# Autodesk Inventor assembly: UM gantry
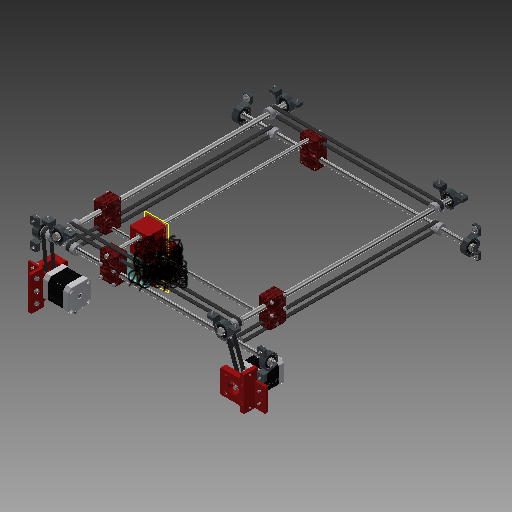
[picture p0: Inventor's stored thumbnail of the model, 512x512]
Saved by Autodesk Inventor 2018.1 (Build 221171000, 171)
## iProperties
Part Number: UM gantry
Material: Generisch
Document SubType Name: Assembly
Designer: Till
Author: Till
## Documents named in this file (18)
- C:\Users\tillm\Dropbox\DIY\CoreBot\UM gantry.iam
- C:\Users\tillm\Dropbox\DIY\CAD\KP08\KP08.iam
- C:\Users\tillm\Dropbox\DIY\CoreBot\CAD Parts\8mm hardened rod.ipt
- C:\Users\tillm\Dropbox\DIY\CoreBot\sliding block.iam
- C:\Users\tillm\Dropbox\DIY\CoreBot\CAD Parts\DriveLine 8x400mm.ipt
- C:\Users\tillm\Dropbox\DIY\CoreBot\CAD Parts\DriveLine 8x350mm.ipt
- C:\Users\tillm\Dropbox\DIY\CoreBot\CAD Parts\1166-B2P-A.ipt
- C:\Users\tillm\Dropbox\DIY\CoreBot\Y belt.ipt
- C:\Users\tillm\Dropbox\DIY\CoreBot\X belt.ipt
- C:\Users\tillm\Dropbox\DIY\CoreBot\CAD Parts\NEMA 17.ipt
- C:\Users\tillm\Dropbox\DIY\CoreBot\CAD Parts\GT2_20teeth_pulley.ipt
- C:\Users\tillm\Dropbox\DIY\CoreBot\CAD Parts\1167-B2P-A (2).ipt
- C:\Users\tillm\Dropbox\DIY\CoreBot\motor belt.ipt
- C:\Users\tillm\Dropbox\DIY\CoreBot\Y motor mount.ipt
- C:\Users\tillm\Dropbox\DIY\CoreBot\X motor mount.ipt
- C:\Users\tillm\Dropbox\DIY\CoreBot\M3 x 10.ipt
- C:\Users\tillm\Dropbox\DIY\CoreBot\CAD Parts\item_0_0_616_29_6rrjpzm9kai2q6ysfss7799ws.ipt
- C:\Users\tillm\Dropbox\DIY\CoreBot\Hotend 2.2.iam
## Components (56 placed, 27 different names)
1. DriveLine 8x400mm:1 — Passend:20, Fluchtend:23, Passend:104
2. DriveLine 8x350mm:1 — Passend:21, Fluchtend:24
3. Hotend 2.2:3 [sub-assembly] — Passend:104, Winkel:12, Fluchtend:106
4. X front right [sub-assembly] — Fluchtend:7, Passend:4, Passend:5, Fluchtend:8, Fluchtend:9, Passend:6, Passend:7, Fluchtend:10, Fluchtend:11, Fluchtend:14, Passend:9, Fluchtend:16, Winkel:3
5. X front left [sub-assembly] — Passend:7, Fluchtend:10, Fluchtend:11, Fluchtend:12, Fluchtend:13, Passend:8, Fluchtend:15, Passend:10, Winkel:4
6. X back right [sub-assembly] — Fluchtend:8, Fluchtend:9, Passend:6, Passend:11, Fluchtend:17, Winkel:7, Fluchtend:43
7. X back left [sub-assembly] — Fluchtend:12, Fluchtend:13, Passend:8
8. Y front right [sub-assembly] — Fluchtend:1, Passend:1, Fluchtend:2, Passend:2, Fluchtend:3, Fluchtend:6, Fluchtend:7, Passend:4, Passend:5, Passend:12, Fluchtend:18, Winkel:1, Passend:71, Fluchtend:42
9. Y front left [sub-assembly] — Passend:2, Fluchtend:3, Fluchtend:4, Passend:3, Fluchtend:5, Fluchtend:6, Passend:13, Fluchtend:19
10. Y back right [sub-assembly] — Fluchtend:1, Passend:1, Fluchtend:2, Fluchtend:44
11. Y back left [sub-assembly] — Fluchtend:4, Passend:3, Fluchtend:5
12. X front — Passend:10, Fluchtend:16, Passend:17, Passend:28, Passend:29, Passend:79
13. X back — Passend:11, Fluchtend:17, Passend:16, Passend:27, Passend:48
14. Y right — Passend:12, Fluchtend:18, Passend:14, Passend:24, Passend:31, Passend:57
15. Y left — Passend:13, Fluchtend:19, Passend:15, Passend:23, Passend:26
16. sliding block:1 [sub-assembly] — Passend:17, Winkel:1, Winkel:2, Passend:21, Fluchtend:24, Winkel:8, Winkel:9, Fluchtend:45, Winkel:11, Passend:78
17. sliding block:2 [sub-assembly] — Passend:16, Winkel:2, Fluchtend:30, Winkel:9, Fluchtend:45, Winkel:10, Winkel:12, Fluchtend:106
18. sliding block:3 [sub-assembly] — Passend:15, Winkel:4, Fluchtend:47, Passend:80
19. sliding block:4 [sub-assembly] — Passend:14, Winkel:3, Passend:20, Fluchtend:23, Fluchtend:28, Fluchtend:47
20. Y belt:1 — Fluchtend:35, Winkel:6, Passend:79, Passend:80
21. Y belt:2 — Passend:35, Winkel:7, Passend:36, Passend:49
22. X belt:1 — Passend:37, Passend:40, Winkel:11, Passend:78
23. X belt:2 — Passend:38, Passend:41, Winkel:10
24. 1167-B2P-A (2):1 — Passend:48, Passend:49, Passend:51, Passend:54
25. 1166-B2P-A:1 — Passend:26, Fluchtend:30, Passend:41, Fluchtend:36
26. 1166-B2P-A:3 — Passend:27, Fluchtend:27, Fluchtend:35
27. 1166-B2P-A:4 — Passend:24, Fluchtend:34, Passend:37, Passend:40
28. 1166-B2P-A:5 — Passend:57, Passend:59, Passend:58
29. 1166-B2P-A:6 — Passend:23, Fluchtend:34
30. 1166-B2P-A:7 — Passend:28, Fluchtend:27
31. 1166-B2P-A:8 — Passend:29, Fluchtend:28, Passend:35, Passend:36
32. 1166-B2P-A:9 — Passend:31, Passend:38, Fluchtend:36
33. item_0_0_616_29_6rrjpzm9kai2q6ysfss7799ws:5 — Fluchtend:56, Passend:103
34. item_0_0_616_29_6rrjpzm9kai2q6ysfss7799ws:6 — Fluchtend:56, Passend:99, Passend:100
35. item_0_0_616_29_6rrjpzm9kai2q6ysfss7799ws:8 — Passend:101
36. M3 x 10:1 — Fluchtend:48, Passend:84, Passend:85
37. M3 x 10:2 — Fluchtend:48, Passend:86
38. M3 x 10:3 — Fluchtend:49, Passend:83
39. M3 x 10:4 — Fluchtend:49, Passend:81, Passend:82
40. GT2_20teeth_pulley:2 — Passend:42, Passend:55, Passend:65
41. NEMA 17:2 — Passend:42, Passend:75, Passend:76, Passend:77
42. motor belt:1 — Passend:51, Passend:54, Passend:55, Passend:65
43. X motor mount:1 — Passend:75, Fluchtend:43, Fluchtend:44, Passend:76, Passend:77, Passend:81, Passend:82, Passend:83, Passend:84, Passend:85, Passend:86, Passend:99, Passend:100, Passend:101, Passend:103
44. item_0_0_616_29_6rrjpzm9kai2q6ysfss7799ws:1 — Fluchtend:55, Passend:94, Passend:95
45. item_0_0_616_29_6rrjpzm9kai2q6ysfss7799ws:2 — Fluchtend:54, Fluchtend:55, Passend:96
46. item_0_0_616_29_6rrjpzm9kai2q6ysfss7799ws:3 — Fluchtend:53, Fluchtend:54, Passend:97
47. item_0_0_616_29_6rrjpzm9kai2q6ysfss7799ws:4 — Fluchtend:53, Passend:98
48. M3 x 10:5 — Fluchtend:50, Passend:93
49. M3 x 10:6 — Fluchtend:50, Passend:91, Passend:92
50. M3 x 10:7 — Fluchtend:51, Passend:89
51. M3 x 10:8 — Fluchtend:51, Fluchtend:52, Passend:90
52. M3 x 10:9 — Fluchtend:52, Passend:87, Passend:88
53. Y motor mount:1 — Passend:71, Fluchtend:42, Passend:72, Passend:73, Passend:74, Winkel:8, Passend:87, Passend:88, Passend:89, Passend:90, Passend:91, Passend:92, Passend:93, Passend:94, Passend:95, Passend:96, Passend:97, Passend:98
54. motor belt:2 — Passend:56, Passend:59, Passend:58, Passend:69
55. GT2_20teeth_pulley:1 — Passend:43, Passend:56, Passend:69
56. NEMA 17:1 — Passend:43, Passend:72, Passend:73, Passend:74
## Relationships (131: Mate 78, Flush 42, Angle 11)
- Fluchtend:1 [Flush]: Y front right ↔ Y back right
- Passend:1 [Mate] (407 mm): Y front right ↔ Y back right
- Fluchtend:2 [Flush]: Y front right ↔ Y back right
- Passend:2 [Mate] (-400 mm): Y front right ↔ Y front left
- Fluchtend:3 [Flush]: Y front right ↔ Y front left
- Fluchtend:4 [Flush]: Y front left ↔ Y back left
- Passend:3 [Mate] (410 mm): Y front left ↔ Y back left
- Fluchtend:5 [Flush]: Y front left ↔ Y back left
- Fluchtend:6 [Flush]: Y front right ↔ Y front left
- Fluchtend:7 [Flush] (-20.1 mm): X front right ↔ Y front right
- Passend:4 [Mate] (23.6 mm): X front right ↔ Y front right
- Passend:5 [Mate] (3.5 mm): X front right ↔ Y front right
- Fluchtend:8 [Flush]: X front right ↔ X back right
- Fluchtend:9 [Flush]: X front right ↔ X back right
- Passend:6 [Mate] (-359.8 mm): X front right ↔ X back right
- Passend:7 [Mate] (407 mm): X front right ↔ X front left
- Fluchtend:10 [Flush]: X front right ↔ X front left
- Fluchtend:11 [Flush]: X front right ↔ X front left
- Fluchtend:12 [Flush]: X front left ↔ X back left
- Fluchtend:13 [Flush]: X front left ↔ X back left
- Passend:8 [Mate] (-359.8 mm): X front left ↔ X back left
- Fluchtend:14 [Flush]: X front right
- Passend:9 [Mate]: X front right
- Fluchtend:15 [Flush]: X front left
- Passend:10 [Mate]: X front left ↔ X front
- Fluchtend:16 [Flush]: X front right ↔ X front
- Passend:11 [Mate]: X back right ↔ X back
- Fluchtend:17 [Flush]: X back right ↔ X back
- Passend:12 [Mate]: Y front right ↔ Y right
- Fluchtend:18 [Flush]: Y front right ↔ Y right
- Passend:13 [Mate]: Y front left ↔ Y left
- Fluchtend:19 [Flush]: Y front left ↔ Y left
- Passend:14 [Mate]: Y right ↔ sliding block:4
- Passend:15 [Mate]: Y left ↔ sliding block:3
- Passend:16 [Mate]: X back ↔ sliding block:2
- Passend:17 [Mate]: X front ↔ sliding block:1
- Winkel:1 [Angle] (0 deg): Y front right ↔ sliding block:1
- Winkel:2 [Angle] (0 deg): sliding block:1 ↔ sliding block:2
- Winkel:3 [Angle] (0 deg): X front right ↔ sliding block:4
- Winkel:4 [Angle] (0 deg): X front left ↔ sliding block:3
- Passend:20 [Mate]: DriveLine 8x400mm:1 ↔ sliding block:4
- Fluchtend:23 [Flush] (-5 mm): DriveLine 8x400mm:1 ↔ sliding block:4
- Passend:21 [Mate]: DriveLine 8x350mm:1 ↔ sliding block:1
- Fluchtend:24 [Flush] (-5 mm): DriveLine 8x350mm:1 ↔ sliding block:1
- Passend:23 [Mate]: Y left ↔ 1166-B2P-A:6
- Passend:24 [Mate]: Y right ↔ 1166-B2P-A:4
- Passend:26 [Mate]: Y left ↔ 1166-B2P-A:1
- Passend:27 [Mate]: X back ↔ 1166-B2P-A:3
- Passend:28 [Mate]: X front ↔ 1166-B2P-A:7
- Passend:29 [Mate]: X front ↔ 1166-B2P-A:8
- Passend:31 [Mate]: Y right ↔ 1166-B2P-A:9
- Fluchtend:34 [Flush]: 1166-B2P-A:4 ↔ 1166-B2P-A:6
- Fluchtend:27 [Flush]: 1166-B2P-A:3 ↔ 1166-B2P-A:7
- Fluchtend:28 [Flush]: sliding block:4 ↔ 1166-B2P-A:8
- Fluchtend:30 [Flush]: sliding block:2 ↔ 1166-B2P-A:1
- Fluchtend:35 [Flush]: Y belt:1 ↔ 1166-B2P-A:3
- Winkel:6 [Angle] (0 deg): Y belt:1
- Passend:35 [Mate]: Y belt:2 ↔ 1166-B2P-A:8
- Winkel:7 [Angle] (0 deg): X back right ↔ Y belt:2
- Passend:36 [Mate]: Y belt:2 ↔ 1166-B2P-A:8
- Passend:37 [Mate]: X belt:1 ↔ 1166-B2P-A:4
- Passend:38 [Mate]: X belt:2 ↔ 1166-B2P-A:9
- Passend:41 [Mate]: X belt:2 ↔ 1166-B2P-A:1
- Passend:40 [Mate]: X belt:1 ↔ 1166-B2P-A:4
- Fluchtend:36 [Flush]: 1166-B2P-A:1 ↔ 1166-B2P-A:9
- Passend:42 [Mate]: GT2_20teeth_pulley:2 ↔ NEMA 17:2
- Passend:43 [Mate]: GT2_20teeth_pulley:1 ↔ NEMA 17:1
- Passend:48 [Mate]: X back ↔ 1167-B2P-A (2):1
- Passend:49 [Mate]: Y belt:2 ↔ 1167-B2P-A (2):1
- Passend:51 [Mate]: 1167-B2P-A (2):1 ↔ motor belt:1
- Passend:54 [Mate] (0.5 mm): 1167-B2P-A (2):1 ↔ motor belt:1
- Passend:55 [Mate]: GT2_20teeth_pulley:2 ↔ motor belt:1
- Passend:56 [Mate]: motor belt:2 ↔ GT2_20teeth_pulley:1
- Passend:57 [Mate]: Y right ↔ 1166-B2P-A:5
- Passend:59 [Mate]: 1166-B2P-A:5 ↔ motor belt:2
- Passend:58 [Mate]: 1166-B2P-A:5 ↔ motor belt:2
- Passend:65 [Mate] (1.5 mm): GT2_20teeth_pulley:2 ↔ motor belt:1
- Passend:69 [Mate] (1.5 mm): motor belt:2 ↔ GT2_20teeth_pulley:1
- Passend:71 [Mate] (3.5 mm): Y front right ↔ Y motor mount:1
- Fluchtend:42 [Flush]: Y front right ↔ Y motor mount:1
- Passend:72 [Mate]: Y motor mount:1 ↔ NEMA 17:1
- Passend:73 [Mate]: Y motor mount:1 ↔ NEMA 17:1
- Passend:74 [Mate]: Y motor mount:1 ↔ NEMA 17:1
- Passend:75 [Mate]: NEMA 17:2 ↔ X motor mount:1
- Fluchtend:43 [Flush] (-20.1 mm): X back right ↔ X motor mount:1
- Fluchtend:44 [Flush]: Y back right ↔ X motor mount:1
- Passend:76 [Mate]: NEMA 17:2 ↔ X motor mount:1
- Passend:77 [Mate]: NEMA 17:2 ↔ X motor mount:1
- Winkel:8 [Angle] (0 deg): sliding block:1 ↔ Y motor mount:1
- Winkel:9 [Angle] (180 deg): sliding block:1 ↔ sliding block:2
- Fluchtend:45 [Flush]: sliding block:1 ↔ sliding block:2
- Winkel:10 [Angle] (0 deg): sliding block:2 ↔ X belt:2
- Winkel:11 [Angle] (0 deg): sliding block:1 ↔ X belt:1
- Passend:78 [Mate]: sliding block:1 ↔ X belt:1
- Fluchtend:47 [Flush]: sliding block:3 ↔ sliding block:4
- Passend:79 [Mate]: X front ↔ Y belt:1
- Passend:80 [Mate]: sliding block:3 ↔ Y belt:1
- Fluchtend:48 [Flush]: M3 x 10:1 ↔ M3 x 10:2
- Fluchtend:49 [Flush]: M3 x 10:3 ↔ M3 x 10:4
- Passend:81 [Mate]: M3 x 10:4 ↔ X motor mount:1
- Passend:82 [Mate]: M3 x 10:4 ↔ X motor mount:1
- Passend:83 [Mate]: M3 x 10:3 ↔ X motor mount:1
- Passend:84 [Mate]: M3 x 10:1 ↔ X motor mount:1
- Passend:85 [Mate]: M3 x 10:1 ↔ X motor mount:1
- Passend:86 [Mate]: M3 x 10:2 ↔ X motor mount:1
- Fluchtend:50 [Flush]: M3 x 10:5 ↔ M3 x 10:6
- Fluchtend:51 [Flush]: M3 x 10:7 ↔ M3 x 10:8
- Fluchtend:52 [Flush]: M3 x 10:8 ↔ M3 x 10:9
- Passend:87 [Mate]: M3 x 10:9 ↔ Y motor mount:1
- Passend:88 [Mate]: M3 x 10:9 ↔ Y motor mount:1
- Passend:89 [Mate]: M3 x 10:7 ↔ Y motor mount:1
- Passend:90 [Mate]: M3 x 10:8 ↔ Y motor mount:1
- Passend:91 [Mate]: M3 x 10:6 ↔ Y motor mount:1
- Passend:92 [Mate]: M3 x 10:6 ↔ Y motor mount:1
- Passend:93 [Mate]: M3 x 10:5 ↔ Y motor mount:1
- Fluchtend:53 [Flush]: item_0_0_616_29_6rrjpzm9kai2q6ysfss7799ws:3 ↔ item_0_0_616_29_6rrjpzm9kai2q6ysfss7799ws:4
- Fluchtend:54 [Flush]: item_0_0_616_29_6rrjpzm9kai2q6ysfss7799ws:2 ↔ item_0_0_616_29_6rrjpzm9kai2q6ysfss7799ws:3
- Fluchtend:55 [Flush]: item_0_0_616_29_6rrjpzm9kai2q6ysfss7799ws:1 ↔ item_0_0_616_29_6rrjpzm9kai2q6ysfss7799ws:2
- Passend:94 [Mate]: item_0_0_616_29_6rrjpzm9kai2q6ysfss7799ws:1 ↔ Y motor mount:1
- Passend:95 [Mate]: item_0_0_616_29_6rrjpzm9kai2q6ysfss7799ws:1 ↔ Y motor mount:1
- Passend:96 [Mate]: item_0_0_616_29_6rrjpzm9kai2q6ysfss7799ws:2 ↔ Y motor mount:1
- Passend:97 [Mate]: item_0_0_616_29_6rrjpzm9kai2q6ysfss7799ws:3 ↔ Y motor mount:1
- Passend:98 [Mate]: item_0_0_616_29_6rrjpzm9kai2q6ysfss7799ws:4 ↔ Y motor mount:1
- Fluchtend:56 [Flush]: item_0_0_616_29_6rrjpzm9kai2q6ysfss7799ws:5 ↔ item_0_0_616_29_6rrjpzm9kai2q6ysfss7799ws:6
- Passend:99 [Mate]: item_0_0_616_29_6rrjpzm9kai2q6ysfss7799ws:6 ↔ X motor mount:1
- Passend:100 [Mate]: item_0_0_616_29_6rrjpzm9kai2q6ysfss7799ws:6 ↔ X motor mount:1
- Passend:101 [Mate]: item_0_0_616_29_6rrjpzm9kai2q6ysfss7799ws:8 ↔ X motor mount:1
- Passend:103 [Mate]: item_0_0_616_29_6rrjpzm9kai2q6ysfss7799ws:5 ↔ X motor mount:1
- Passend:104 [Mate]: DriveLine 8x400mm:1 ↔ Hotend 2.2:3
- Winkel:12 [Angle] (0 deg): Hotend 2.2:3 ↔ sliding block:2
- Fluchtend:106 [Flush] (2.5 mm): Hotend 2.2:3 ↔ sliding block:2
